# Autodesk Inventor assembly: ASY ДМФ 0100 Барабан v2.1
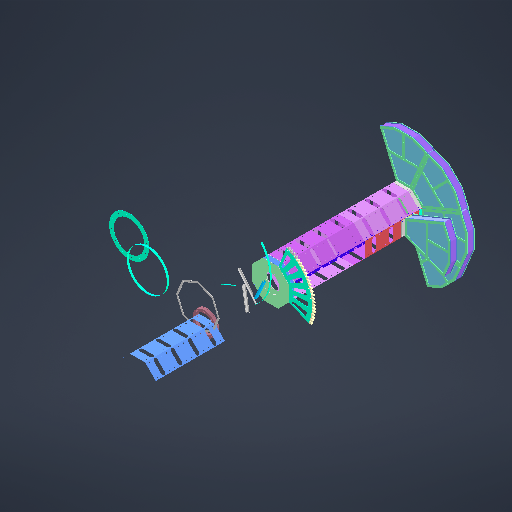
[picture p0: Inventor's stored thumbnail of the model, 512x512]
Saved by Autodesk Inventor 2026.2 (Build 302298010, 298A)
## iProperties
Created: 2024-04-28
Part Number: ASY ДМФ 0100 Барабан v2.1
Document SubType Name: Assembly
Designer: pokla
Author: pokla
## Documents named in this file (24)
- C:\Users\admin\Documents\Inventor\DMF-Disk-Micro-Filter\Барабан v2.1\ASY ДМФ 0100 Барабан v2.1.iam
- C:\Users\admin\Documents\Inventor\DMF-Disk-Micro-Filter\Барабан v2.1\DMF 01 21 Барабан торец НОС v2.1.ipt
- C:\Users\admin\Documents\Inventor\DMF-Disk-Micro-Filter\Барабан v2.1\DMF 01 13 Барабан Лист лев брт v2.1.ipt
- C:\Users\admin\Documents\Inventor\DMF-Disk-Micro-Filter\Барабан v2.1\DMF 01 14 Барабан Лист прав брт v2.1.ipt
- C:\Users\admin\Documents\Inventor\DMF-Disk-Micro-Filter\Барабан v2.1\DMF 01 31 Барабан Опорное кольцо НОС v2.1.ipt
- C:\Users\admin\Documents\Inventor\DMF-Disk-Micro-Filter\Барабан v2.1\DMF 01 17 опора крышки v2.1.ipt
- C:\Users\admin\Documents\Inventor\DMF-Disk-Micro-Filter\Барабан v2.1\DMF 000 размеры v2.1.ipt
- C:\Users\admin\Documents\Inventor\DMF-Disk-Micro-Filter\Барабан v2.1\DMF 01 12 Барабан усилитель v2.1.ipt
- C:\Users\admin\Documents\Inventor\DMF-Disk-Micro-Filter\Барабан v2.1\ASY DMF 010 cap v2.1.iam
- C:\Users\admin\Documents\Inventor\DMF-Disk-Micro-Filter\Барабан v2.1\DMF 01 32 Барабан Опорное кольцо КОРМА v2.1.ipt
- C:\Users\admin\Documents\Inventor\DMF-Disk-Micro-Filter\Барабан v2.1\DMF 01 22 Барабан торец КОРМА v2.1.ipt
- C:\Users\admin\Documents\Inventor\DMF-Disk-Micro-Filter\Барабан v2.1\ASY DMF filter package v2.1.iam
- C:\Users\admin\Documents\Inventor\DMF-Disk-Micro-Filter\Барабан v2.1\DMF 2.1 01 43 Gear rim 3.ipt
- C:\Users\admin\Documents\Inventor\DMF-Disk-Micro-Filter\Барабан v2.1\DMF 2.1 01 44 Gear rim 4.ipt
- C:\Users\admin\Documents\Inventor\DMF-Disk-Micro-Filter\Барабан v2.1\DMF 2.1 01 45 Gear ring 5.ipt
- C:\Users\admin\Documents\Inventor\DMF-Disk-Micro-Filter\Барабан v2.1\DMF 2.1 01 46 Gear axis wheel 6.ipt
- C:\Users\admin\Documents\Inventor\DMF-Disk-Micro-Filter\Барабан v2.1\DMF 01 13 Барабан усилитель v2.1.ipt
- C:\Users\admin\Documents\Inventor\DMF-Disk-Micro-Filter\шестерни 06.09.2025\DMF sector big gear 2.1.ipt
- C:\Users\admin\Documents\Inventor\DMF-Disk-Micro-Filter\Барабан v2.1\DMF 01 15 drum sheet 1.ipt
- C:\Users\admin\Documents\Inventor\DMF-Disk-Micro-Filter\ДМФ 01 12 Барабан усилитель.ipt
- C:\Users\admin\Documents\Inventor\DMF-Disk-Micro-Filter\ДМФ 01 15 Барабан усилитель борта.ipt
- C:\Users\admin\Documents\Inventor\DMF-Disk-Micro-Filter\Барабан v2.1\DMF 2.1 Пластина паза маленькая.ipt
- C:\Users\admin\Documents\Inventor\DMF-Disk-Micro-Filter\Барабан v2.1\DMF 2.1 Пластина паза большая.ipt
- C:\Users\admin\Documents\Inventor\DMF-Disk-Micro-Filter\Барабан v2.1\DMF 01 11 cylinder sheet cap v2.1.ipt
## Components (42 placed, 31 different names)
1. DMF 000 размеры v2.1.ipt:1
2. DMF 01 21 Барабан торец НОС v2.1.ipt:1 — Rigid:115, Rigid:120
3. DMF 01 31 Барабан Опорное кольцо НОС v2.1.ipt:1
4. DMF 01 32 Барабан Опорное кольцо КОРМА v2.1.ipt:1 — Rigid:20
5. DMF 01 22 Барабан торец КОРМА v2.1.ipt:1 — Rigid:20, Rigid:51, Mate:37, Rigid:97, Mate:46, Mate:50, Flush:36, Mate:51
6. DMF 01 13 Барабан Лист лев брт v2.1.ipt:1 — Rigid:51, Rigid:98
7. DMF 01 14 Барабан Лист прав брт v2.1.ipt:1
8. DMF 01 17 опора крышки v2.1.ipt:1 — Mate:37, Mate:46, Mate:47, Mate:48, Rigid:112
9. DMF 01 11 cylinder sheet cap v2.1.ipt:1 — Mate:47, Rigid:100
10. ASY DMF 010 cap v2.1.iam:1 [sub-assembly]
11. DMF 2.1 01 45 Gear ring 5.ipt:1
12. DMF 2.1 01 46 Gear axis wheel 6.ipt:1
13. DMF 2.1 01 44 Gear rim 4.ipt:1 — Rigid:110
14. DMF 01 15 drum sheet 1.ipt:1 — Rigid:118
15. ДМФ 01 12 Барабан усилитель.ipt:2 — Rigid:57, Rigid:89
16. ДМФ 01 15 Барабан усилитель борта.ipt:4 — Rigid:57
17. ДМФ 01 12 Барабан усилитель:3 — Rigid:89
18. ДМФ 01 15 Барабан усилитель борта:5
19. ДМФ 01 15 Барабан усилитель борта:6
20. DMF 01 12 Барабан усилитель v2.1.ipt:2
21. DMF 01 13 Барабан усилитель v2.1.ipt:2
22. DMF 2.1 Пластина паза маленькая.ipt:1
23. DMF 2.1 Пластина паза большая:1 — Rigid:110
24. ASY DMF filter package v2.1.iam:1 [sub-assembly]
25. DMF sector big gear 2.1.ipt:1 — Rigid:104, Rigid:117
26. ASY DMF filter package v2.1:2 [sub-assembly]
27. ASY DMF filter package v2.1:3 [sub-assembly] — Rigid:113
28. DMF 01 13 Барабан Лист лев брт v2.1:2 — Rigid:97, Rigid:99, Mate:48, Rigid:113, Rigid:114
29. DMF 01 13 Барабан Лист лев брт v2.1:3 — Rigid:98
30. DMF 01 13 Барабан Лист лев брт v2.1:4 — Rigid:99, Rigid:115
31. DMF sector big gear 2.1:2 — Rigid:104, Rigid:105
32. DMF sector big gear 2.1:3 — Rigid:105, Rigid:106
33. DMF sector big gear 2.1:4 — Rigid:106, Rigid:107
34. DMF sector big gear 2.1:5 — Rigid:107, Rigid:108
35. DMF sector big gear 2.1:6 — Rigid:108
36. DMF 01 17 опора крышки v2.1:4 — Rigid:112
37. DMF 2.1 01 43 Gear rim 3.ipt:2 — Rigid:117, Flush:37, Mate:52, Mate:53
38. ASY DMF filter package v2.1:5 [sub-assembly] — Rigid:100
39. ASY DMF filter package v2.1:4 [sub-assembly] — Rigid:114
40. DMF 01 21 Барабан торец НОС v2.1:3 — Rigid:118, Rigid:119, Rigid:120
41. DMF 01 15 drum sheet 1:2 — Rigid:119, Rigid:121, Mate:52, Mate:53
42. DMF 01 21 Барабан торец НОС v2.1:4 — Rigid:121, Flush:37
## Relationships (40: WeldJoint 27, Mate 9, Flush 4)
- Rigid:20 [WeldJoint]: DMF 01 32 Барабан Опорное кольцо КОРМА v2.1.ipt:1 ↔ DMF 01 22 Барабан торец КОРМА v2.1.ipt:1
- Rigid:51 [WeldJoint]: DMF 01 22 Барабан торец КОРМА v2.1.ipt:1 ↔ DMF 01 13 Барабан Лист лев брт v2.1.ipt:1
- Mate:37: DMF 01 22 Барабан торец КОРМА v2.1.ipt:1 ↔ DMF 01 17 опора крышки v2.1.ipt:1
- Rigid:57 [WeldJoint]: ДМФ 01 12 Барабан усилитель.ipt:2 ↔ ДМФ 01 15 Барабан усилитель борта.ipt:4
- [Mate]: DMF 01 22 Барабан торец КОРМА v2.1.ipt:1 ↔ DMF 01 11 cylinder sheet cap v2.1.ipt:1
- [Flush]: DMF 01 22 Барабан торец КОРМА v2.1.ipt:1 ↔ DMF 01 11 cylinder sheet cap v2.1.ipt:1
- [Flush]: DMF 01 22 Барабан торец КОРМА v2.1.ipt:1 ↔ DMF 01 11 cylinder sheet cap v2.1.ipt:1
- [WeldJoint]: ДМФ 01 12 Барабан усилитель:3 ↔ ДМФ 01 15 Барабан усилитель борта:5
- [WeldJoint]: ДМФ 01 12 Барабан усилитель:3 ↔ ДМФ 01 15 Барабан усилитель борта:6
- Rigid:89 [WeldJoint]: ДМФ 01 12 Барабан усилитель.ipt:2 ↔ ДМФ 01 12 Барабан усилитель:3
- [WeldJoint]: DMF 01 11 cylinder sheet cap v2.1.ipt:1 ↔ ASY DMF filter package v2.1.iam:1
- [WeldJoint]: DMF 01 11 cylinder sheet cap v2.1.ipt:1 ↔ ASY DMF filter package v2.1:2
- Rigid:97 [WeldJoint]: DMF 01 22 Барабан торец КОРМА v2.1.ipt:1 ↔ DMF 01 13 Барабан Лист лев брт v2.1:2
- Rigid:98 [WeldJoint]: DMF 01 13 Барабан Лист лев брт v2.1.ipt:1 ↔ DMF 01 13 Барабан Лист лев брт v2.1:3
- Rigid:99 [WeldJoint]: DMF 01 13 Барабан Лист лев брт v2.1:2 ↔ DMF 01 13 Барабан Лист лев брт v2.1:4
- Mate:46: DMF 01 22 Барабан торец КОРМА v2.1.ipt:1 ↔ DMF 01 17 опора крышки v2.1.ipt:1
- Mate:47: DMF 01 17 опора крышки v2.1.ipt:1 ↔ DMF 01 11 cylinder sheet cap v2.1.ipt:1
- Mate:48: DMF 01 17 опора крышки v2.1.ipt:1 ↔ DMF 01 13 Барабан Лист лев брт v2.1:2
- Rigid:100 [WeldJoint]: DMF 01 11 cylinder sheet cap v2.1.ipt:1 ↔ ASY DMF filter package v2.1:5
- Rigid:104 [WeldJoint]: DMF sector big gear 2.1.ipt:1 ↔ DMF sector big gear 2.1:2
- Rigid:105 [WeldJoint]: DMF sector big gear 2.1:2 ↔ DMF sector big gear 2.1:3
- Rigid:106 [WeldJoint]: DMF sector big gear 2.1:3 ↔ DMF sector big gear 2.1:4
- Rigid:107 [WeldJoint]: DMF sector big gear 2.1:4 ↔ DMF sector big gear 2.1:5
- Rigid:108 [WeldJoint]: DMF sector big gear 2.1:5 ↔ DMF sector big gear 2.1:6
- Rigid:110 [WeldJoint]: DMF 2.1 01 44 Gear rim 4.ipt:1 ↔ DMF 2.1 Пластина паза большая:1
- Rigid:112 [WeldJoint]: DMF 01 17 опора крышки v2.1.ipt:1 ↔ DMF 01 17 опора крышки v2.1:4
- Mate:50: DMF 01 22 Барабан торец КОРМА v2.1.ipt:1
- Flush:36: DMF 01 22 Барабан торец КОРМА v2.1.ipt:1
- Mate:51: DMF 01 22 Барабан торец КОРМА v2.1.ipt:1
- Rigid:113 [WeldJoint]: ASY DMF filter package v2.1:3 ↔ DMF 01 13 Барабан Лист лев брт v2.1:2
- Rigid:114 [WeldJoint]: DMF 01 13 Барабан Лист лев брт v2.1:2 ↔ ASY DMF filter package v2.1:4
- Rigid:115 [WeldJoint]: DMF 01 21 Барабан торец НОС v2.1.ipt:1 ↔ DMF 01 13 Барабан Лист лев брт v2.1:4
- Rigid:117 [WeldJoint]: DMF sector big gear 2.1.ipt:1 ↔ DMF 2.1 01 43 Gear rim 3.ipt:2
- Rigid:118 [WeldJoint]: DMF 01 15 drum sheet 1.ipt:1 ↔ DMF 01 21 Барабан торец НОС v2.1:3
- Rigid:119 [WeldJoint]: DMF 01 21 Барабан торец НОС v2.1:3 ↔ DMF 01 15 drum sheet 1:2
- Rigid:120 [WeldJoint]: DMF 01 21 Барабан торец НОС v2.1.ipt:1 ↔ DMF 01 21 Барабан торец НОС v2.1:3
- Rigid:121 [WeldJoint]: DMF 01 15 drum sheet 1:2 ↔ DMF 01 21 Барабан торец НОС v2.1:4
- Flush:37: DMF 2.1 01 43 Gear rim 3.ipt:2 ↔ DMF 01 21 Барабан торец НОС v2.1:4
- Mate:52: DMF 2.1 01 43 Gear rim 3.ipt:2 ↔ DMF 01 15 drum sheet 1:2
- Mate:53: DMF 2.1 01 43 Gear rim 3.ipt:2 ↔ DMF 01 15 drum sheet 1:2
## Named parameters: d460_d378 = 0 mm, d461_d379 = 0 mm
